# Autodesk Inventor assembly: DCMotorAssembly
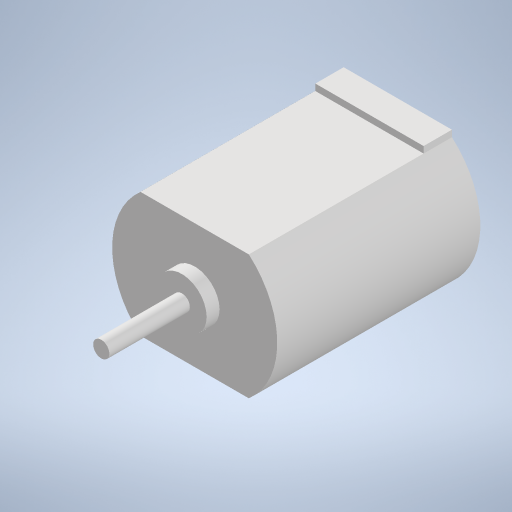
[picture p0: Inventor's stored thumbnail of the model, 512x512]
Saved by Autodesk Inventor 2023 (Build 270158000, 158)
## iProperties
Created: 2023-03-13
Part Number: DCMotorAssembly
Document SubType Name: Assembly
Designer: czapa
Author: czapa
## Documents named in this file (3)
- C:\Users\czapa\OneDrive\Documents\GitHub\S.P.I.C.E\3D Models\DCMotorAssembly.iam
- C:\Users\czapa\OneDrive\Documents\GitHub\S.P.I.C.E\3D Models\DCMotor.ipt
- C:\Users\czapa\OneDrive\Documents\GitHub\S.P.I.C.E\3D Models\DCMotorShaft.ipt
## Components (2 placed, 2 different names)
1. DCMotor:1 — Mate:1, Mate:2
2. DCMotorShaft:1 — Mate:1, Mate:2
## Relationships (2: Mate 2)
- Mate:1: DCMotor:1 ↔ DCMotorShaft:1
- Mate:2: DCMotor:1 ↔ DCMotorShaft:1
